# Autodesk Inventor assembly: Watercooling_Rad
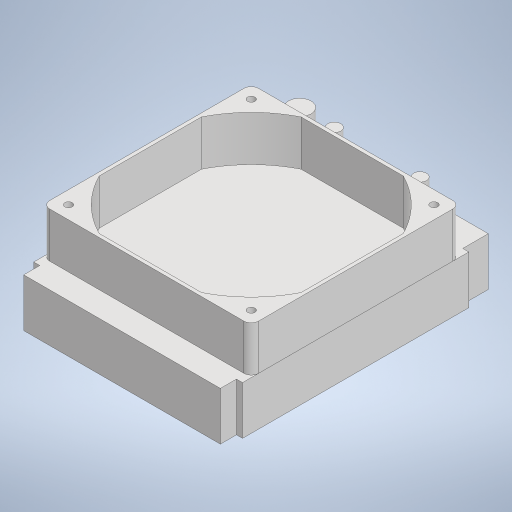
[picture p0: Inventor's stored thumbnail of the model, 512x512]
Saved by Autodesk Inventor 2023 (Build 270158000, 158)
## iProperties
Created: 2023-08-19
Part Number: Watercooling_Rad
Document SubType Name: Assembly
Designer: plebbb
Author: plebbb
## Documents named in this file (3)
- D:\Users\plebbb\Desktop\CNC_Project\Watercooling_Rad.iam
- D:\Users\plebbb\Desktop\CNC_Project\120mm_fan.ipt
- D:\Users\plebbb\Desktop\CNC_Project\Radiator.ipt
## Components (2 placed, 2 different names)
1. 120mm_fan:1 — Mate:1, Mate:2, Mate:3
2. Radiator:1 — Mate:1, Mate:2, Mate:3
## Relationships (3: Mate 3)
- Mate:1: 120mm_fan:1 ↔ Radiator:1
- Mate:2: 120mm_fan:1 ↔ Radiator:1
- Mate:3: 120mm_fan:1 ↔ Radiator:1
